# Autodesk Inventor assembly: Assieme maschera
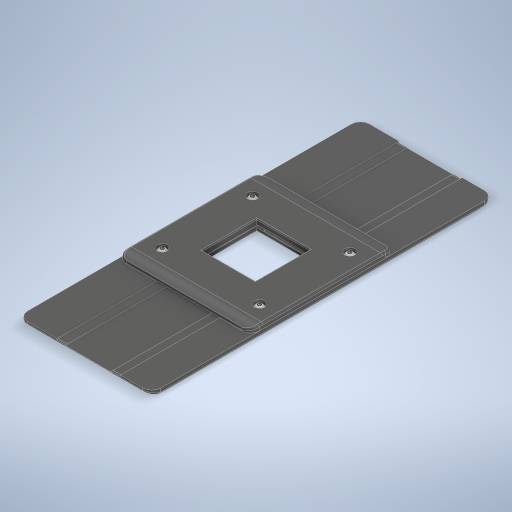
[picture p0: Inventor's stored thumbnail of the model, 512x512]
Saved by Autodesk Inventor 2023 (Build 270158000, 158)
## iProperties
Created: 2026-01-13
Part Number: Assieme maschera
Document SubType Name: Assembly
Designer: Davide
1_Materiale: − − −
2_Trattamento: − − −
3_Disegnato: D. Mitidieri
4_Controllato: C. Pirrottina
5_Approvato: S. Musella
Author: Davide
## Documents named in this file (5)
- C:\Users\Davide\Documents\GitHub\Film-carriers\126\IDW\Assembly.iam
- C:\Users\Davide\Documents\GitHub\Film-carriers\126\IDW\Base.ipt
- C:\Users\Davide\Documents\GitHub\Film-carriers\126\IDW\Mask.ipt
- C:\Users\Davide\Documents\GitHub\Film-carriers\126\IDW\Fasteners\Nut.ipt
- C:\Users\Davide\Documents\GitHub\Film-carriers\126\IDW\Fasteners\Bolt ISO 7380.ipt
## Components (10 placed, 4 different names)
1. Base:1 — Allineato:2, Coincidente:1, Coincidente:2, Inserimento:9, Inserimento:10, Inserimento:11, Inserimento:12
2. Mask:1 — Allineato:2, Coincidente:1, Coincidente:2, Inserimento:5, Inserimento:6, Inserimento:7, Inserimento:8
3. Nut:1 — Inserimento:11
4. Nut:2 — Inserimento:12
5. Nut:3 — Inserimento:9
6. Nut:4 — Inserimento:10
7. Bolt ISO 7380:1 — Inserimento:5
8. Bolt ISO 7380:2 — Inserimento:7
9. Bolt ISO 7380:3 — Inserimento:6
10. Bolt ISO 7380:4 — Inserimento:8
## Relationships (11: Insert 8, Mate 2, Flush 1)
- Allineato:2 [Flush]: Base:1 ↔ Mask:1
- Coincidente:1 [Mate]: Base:1 ↔ Mask:1
- Coincidente:2 [Mate]: Base:1 ↔ Mask:1
- Inserimento:5: Mask:1 ↔ Bolt ISO 7380:1
- Inserimento:6: Mask:1 ↔ Bolt ISO 7380:3
- Inserimento:7: Mask:1 ↔ Bolt ISO 7380:2
- Inserimento:8: Mask:1 ↔ Bolt ISO 7380:4
- Inserimento:9: Base:1 ↔ Nut:3
- Inserimento:10: Base:1 ↔ Nut:4
- Inserimento:11: Base:1 ↔ Nut:1
- Inserimento:12: Base:1 ↔ Nut:2
